# Autodesk Inventor assembly: ensamble resistencias
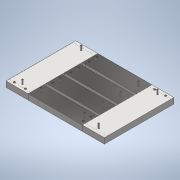
[picture p0: Inventor's stored thumbnail of the model, 180x180]
Saved by Autodesk Inventor 2021 (Build 250183000, 183)
## iProperties
Created: 2021-04-16
Part Number: ensamble resistencias
Document SubType Name: Assembly
Designer: Leonardo Fabio Mercado Benítez
Author: Leonardo Fabio Mercado Benítez
## Documents named in this file (3)
- C:\Users\leo7s\Documents\Universidad\04 PAI\03 Proyecto\03 Github\Proyecto_PAI_2021\01 CAD\ensamble resistencias.iam
- C:\Users\leo7s\Documents\Universidad\04 PAI\03 Proyecto\03 Github\Proyecto_PAI_2021\01 CAD\resistencia_cuarzo_550W.ipt
- C:\Users\leo7s\Documents\Universidad\04 PAI\03 Proyecto\03 Github\Proyecto_PAI_2021\01 CAD\resistencia_cuarzo_250-300W.ipt
## Components (6 placed, 2 different names)
1. resistencia_cuarzo_550W:1 — Nivelación:1, Nivelación:2, Coincidencia:1, Nivelación:3, Nivelación:4, Coincidencia:2, Nivelación:5, Nivelación:6, Coincidencia:3, Coincidencia:4
2. resistencia_cuarzo_550W:2 — Nivelación:7, Nivelación:8, Coincidencia:7
3. resistencia_cuarzo_250-300W:1 — Nivelación:3, Nivelación:4, Coincidencia:2, Coincidencia:6, Nivelación:7, Nivelación:8, Coincidencia:7
4. resistencia_cuarzo_250-300W:2 — Nivelación:6, Coincidencia:4, Coincidencia:6
5. resistencia_cuarzo_250-300W:3 — Nivelación:5, Coincidencia:3, Coincidencia:5
6. resistencia_cuarzo_250-300W:4 — Nivelación:1, Nivelación:2, Coincidencia:1, Coincidencia:5
## Relationships (15: Flush 8, Mate 7)
- Nivelación:1 [Flush]: resistencia_cuarzo_550W:1 ↔ resistencia_cuarzo_250-300W:4
- Nivelación:2 [Flush]: resistencia_cuarzo_550W:1 ↔ resistencia_cuarzo_250-300W:4
- Coincidencia:1 [Mate]: resistencia_cuarzo_550W:1 ↔ resistencia_cuarzo_250-300W:4
- Nivelación:3 [Flush]: resistencia_cuarzo_550W:1 ↔ resistencia_cuarzo_250-300W:1
- Nivelación:4 [Flush]: resistencia_cuarzo_550W:1 ↔ resistencia_cuarzo_250-300W:1
- Coincidencia:2 [Mate]: resistencia_cuarzo_550W:1 ↔ resistencia_cuarzo_250-300W:1
- Nivelación:5 [Flush]: resistencia_cuarzo_550W:1 ↔ resistencia_cuarzo_250-300W:3
- Nivelación:6 [Flush]: resistencia_cuarzo_550W:1 ↔ resistencia_cuarzo_250-300W:2
- Coincidencia:3 [Mate]: resistencia_cuarzo_550W:1 ↔ resistencia_cuarzo_250-300W:3
- Coincidencia:4 [Mate]: resistencia_cuarzo_550W:1 ↔ resistencia_cuarzo_250-300W:2
- Coincidencia:5 [Mate] (11.67 mm): resistencia_cuarzo_250-300W:3 ↔ resistencia_cuarzo_250-300W:4
- Coincidencia:6 [Mate] (11.67 mm): resistencia_cuarzo_250-300W:1 ↔ resistencia_cuarzo_250-300W:2
- Nivelación:7 [Flush]: resistencia_cuarzo_550W:2 ↔ resistencia_cuarzo_250-300W:1
- Nivelación:8 [Flush]: resistencia_cuarzo_550W:2 ↔ resistencia_cuarzo_250-300W:1
- Coincidencia:7 [Mate]: resistencia_cuarzo_550W:2 ↔ resistencia_cuarzo_250-300W:1
